# Autodesk Inventor assembly: inner_MIR
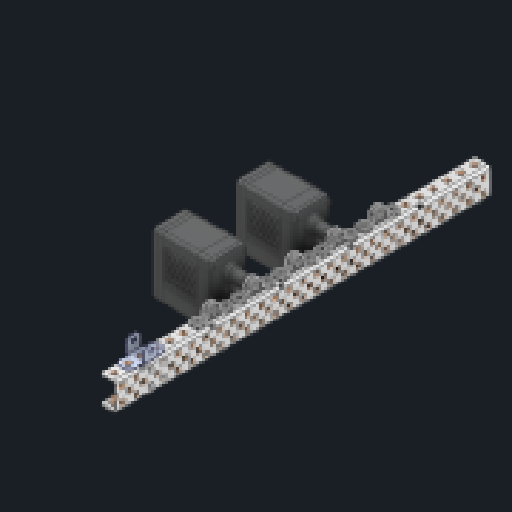
[picture p0: Inventor's stored thumbnail of the model, 512x512]
Saved by Autodesk Inventor 2024 (Build 280153000, 153)
## iProperties
Created: 2023-08-15
Part Number: inner_MIR
Document SubType Name: Assembly
Designer: avere
Author: avere
## Documents named in this file (14)
- D:\cad\scrap_v0.1\chassis\mirrored_parts\inner_MIR.iam
- D:\cad\scrap_v0.1\chassis\mirrored_parts\Alu C 1x2x1x27_MIR.ipt
- D:\cad\scrap_v0.1\chassis\mirrored_parts\LS Pillow Bearing Block_MIR.ipt
- D:\cad\scrap_v0.1\chassis\mirrored_parts\V5 Motor_MIR.ipt
- D:\cad\VEX-CAD-Inventor-1.41\Motion\Spacers\Spacer Nylon .375 OD\NSpacer .375 OD x .125.ipt
- D:\cad\VEX-CAD-Inventor-1.41\Motion\Spacers\Spacer Nylon .375 OD\NSpacer .375 OD x .500.ipt
- D:\cad\scrap_v0.1\chassis\mirrored_parts\4-Post Hex Nut Retainer_MIR.ipt
- D:\cad\scrap_v0.1\chassis\mirrored_parts\Bearing Flat_MIR1.ipt
- D:\cad\scrap_v0.1\chassis\mirrored_parts\C Channel Coupler_MIR.ipt
- D:\cad\VEX-CAD-Inventor-1.41\Motion\Gears\LS 12T Gear Steel.ipt
- D:\cad\VEX-CAD-Inventor-1.41\Motion\Shaft LS\Bearing Flat Low Profile.ipt
- D:\cad\VEX-CAD-Inventor-1.41\Motion\Spacers\Spacer Nylon .375 OD\NSpacer .375 OD x .250.ipt
- D:\cad\VEX-CAD-Inventor-1.41\Motion\Spacers\Spacer Nylon .375 OD.ipt
- D:\cad\VEX-CAD-Inventor-1.41\Motion\Pneumatics\Cylinder Rod Pivot.ipt
## Components (21 placed, 12 different names)
1. Alu C 1x2x1x27_MIR:1 — Mate:15, Insert:30, Mate:16, Insert:35, Mate:17, Insert:36, Insert:31, Mate:15, Insert:32, Mate:17, Insert:36, Mate:19, Insert:37, Mate:20, Insert:38, Insert:39, Insert:40, Mate:21, Mate:22, Mate:23, Insert:46, Mate:24, Insert:47, Insert:48, Mate:25
2. LS Pillow Bearing Block_MIR:1 — Insert:36, Mate:19
3. 4-Post Hex Nut Retainer_MIR:1 — Mate:15, Insert:30
4. Bearing Flat_MIR1:1 — Mate:16, Insert:35
5. C Channel Coupler_MIR:1 — Mate:17, Insert:36
6. LS Pillow Bearing Block_MIR:4 — Insert:37, Mate:20
7. LS 12T Gear Steel:1 — Insert:42
8. LS Pillow Bearing Block_MIR:6 — Insert:31, Mate:15
9. LS Pillow Bearing Block_MIR:7 — Insert:32, Insert:33, Mate:17
10. V5 Motor_MIR:6 — Insert:34, Insert:35
11. NSpacer .375 OD x .125:12 — Insert:33, Insert:34
12. NSpacer .375 OD x .500:13 — Insert:35
13. Bearing Flat Low Profile:1 — Insert:38, Mate:23
14. Bearing Flat Low Profile:2 — Insert:39, Mate:22
15. Bearing Flat Low Profile:4 — Insert:40, Mate:21, Insert:41
16. NSpacer .375 OD x .250:14 — Insert:41, Insert:42
17. LS Pillow Bearing Block_MIR:8 — Insert:46, Mate:24
18. V5 Motor_MIR:7
19. NSpacer .375 OD x .125:15
20. NSpacer .375 OD x .500:16 — Insert:47
21. Cylinder Rod Pivot:1 — Insert:48, Mate:25
## Relationships (33: Insert 21, Mate 12)
- Mate:15: Alu C 1x2x1x27_MIR:1 ↔ 4-Post Hex Nut Retainer_MIR:1
- Insert:30: Alu C 1x2x1x27_MIR:1 ↔ 4-Post Hex Nut Retainer_MIR:1
- Mate:16: Alu C 1x2x1x27_MIR:1 ↔ Bearing Flat_MIR1:1
- Insert:35: Alu C 1x2x1x27_MIR:1 ↔ Bearing Flat_MIR1:1
- Mate:17: Alu C 1x2x1x27_MIR:1 ↔ C Channel Coupler_MIR:1
- Insert:36: Alu C 1x2x1x27_MIR:1 ↔ C Channel Coupler_MIR:1
- Insert:31: Alu C 1x2x1x27_MIR:1 ↔ LS Pillow Bearing Block_MIR:6
- Mate:15: Alu C 1x2x1x27_MIR:1 ↔ LS Pillow Bearing Block_MIR:6
- Insert:32: Alu C 1x2x1x27_MIR:1 ↔ LS Pillow Bearing Block_MIR:7
- Insert:33: LS Pillow Bearing Block_MIR:7 ↔ NSpacer .375 OD x .125:12
- Insert:34: V5 Motor_MIR:6 ↔ NSpacer .375 OD x .125:12
- Insert:35: V5 Motor_MIR:6 ↔ NSpacer .375 OD x .500:13
- Mate:17: Alu C 1x2x1x27_MIR:1 ↔ LS Pillow Bearing Block_MIR:7
- Insert:36: Alu C 1x2x1x27_MIR:1 ↔ LS Pillow Bearing Block_MIR:1
- Mate:19: Alu C 1x2x1x27_MIR:1 ↔ LS Pillow Bearing Block_MIR:1
- Insert:37: Alu C 1x2x1x27_MIR:1 ↔ LS Pillow Bearing Block_MIR:4
- Mate:20: Alu C 1x2x1x27_MIR:1 ↔ LS Pillow Bearing Block_MIR:4
- Insert:38: Alu C 1x2x1x27_MIR:1 ↔ Bearing Flat Low Profile:1
- Insert:39: Alu C 1x2x1x27_MIR:1 ↔ Bearing Flat Low Profile:2
- Insert:40: Alu C 1x2x1x27_MIR:1 ↔ Bearing Flat Low Profile:4
- Mate:21: Alu C 1x2x1x27_MIR:1 ↔ Bearing Flat Low Profile:4
- Mate:22: Alu C 1x2x1x27_MIR:1 ↔ Bearing Flat Low Profile:2
- Mate:23: Alu C 1x2x1x27_MIR:1 ↔ Bearing Flat Low Profile:1
- Insert:41 (1.27 mm): Bearing Flat Low Profile:4 ↔ NSpacer .375 OD x .250:14
- Insert:42: LS 12T Gear Steel:1 ↔ NSpacer .375 OD x .250:14
- [Insert] (3.175 mm): LS Pillow Bearing Block_MIR:8 ↔ V5 Motor_MIR:7
- [Insert]: LS Pillow Bearing Block_MIR:8 ↔ NSpacer .375 OD x .125:15
- [Insert]: V5 Motor_MIR:7 ↔ NSpacer .375 OD x .500:16
- Insert:46: Alu C 1x2x1x27_MIR:1 ↔ LS Pillow Bearing Block_MIR:8
- Mate:24: Alu C 1x2x1x27_MIR:1 ↔ LS Pillow Bearing Block_MIR:8
- Insert:47: Alu C 1x2x1x27_MIR:1 ↔ NSpacer .375 OD x .500:16
- Insert:48: Alu C 1x2x1x27_MIR:1 ↔ Cylinder Rod Pivot:1
- Mate:25: Alu C 1x2x1x27_MIR:1 ↔ Cylinder Rod Pivot:1
## Named parameters: d65_d41_d18 = 3.175 mm, d66_d42_d19 = 0 mm, d67_d43_d21 = 0 mm
